# Autodesk Inventor assembly: wheel
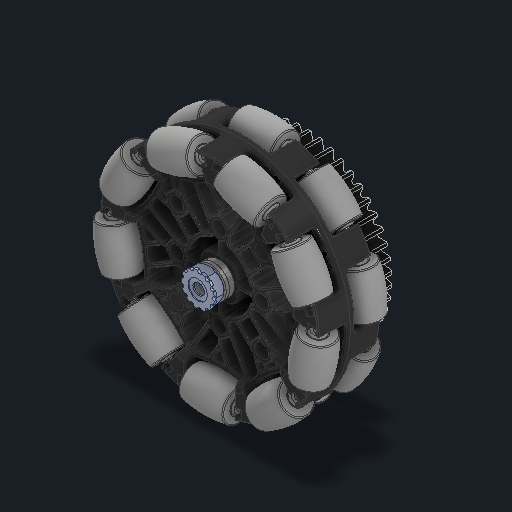
[picture p0: Inventor's stored thumbnail of the model, 512x512]
Saved by Autodesk Inventor 2024 (Build 280153000, 153)
## iProperties
Created: 2024-02-11
Part Number: wheel
Document SubType Name: Assembly
Designer: Averey Ku
Author: Averey Ku
## Documents named in this file (11)
- D:\vex_robotics\hardware\cad\vroomba_v0.1\chassis\drivebay\wheel.iam
- D:\vex_robotics\hardware\cad\VEX-CAD-Inventor-1.41\Motion\Wheels\Omni Wheel\2.75 Omni AS, No Insert.iam
- D:\vex_robotics\hardware\cad\VEX-CAD-Inventor-1.41\Motion\Wheels\Omni Wheel.iam
- D:\vex_robotics\hardware\cad\VEX-CAD-Inventor-1.41\Motion\Spacers\Spacer Nylon .375 OD\NSpacer .375 OD x .250.ipt
- D:\vex_robotics\hardware\cad\VEX-CAD-Inventor-1.41\Motion\Spacers\Spacer Nylon .375 OD.ipt
- D:\vex_robotics\hardware\cad\vroomba_v0.1\custom_parts\LS 48T Gear, No Insert.ipt
- D:\vex_robotics\hardware\cad\VEX-CAD-Inventor-1.41\Motion\Spacers\Washer Teflon\TWasher .375 OD x .04000.ipt
- D:\vex_robotics\hardware\cad\VEX-CAD-Inventor-1.41\Motion\Spacers\Washer Teflon.ipt
- D:\vex_robotics\hardware\cad\VEX-CAD-Inventor-1.41\Motion\Spacers\Washer Steel\SWasher .375 OD x .062500.ipt
- D:\vex_robotics\hardware\cad\VEX-CAD-Inventor-1.41\Motion\Spacers\Washer Steel.ipt
- D:\vex_robotics\hardware\cad\VEX-CAD-Inventor-1.41\Structure\Hardware\Nut Keps.ipt
## Components (7 placed, 6 different names)
1. 2.75 Omni AS, No Insert:1 [sub-assembly] — Insert:1, Insert:2, Insert:6
2. NSpacer .375 OD x .250:1 — Insert:1, Mate:1
3. NSpacer .375 OD x .250:2 — Insert:2, Insert:3
4. LS 48T Gear, No Insert:1 — Insert:3, Mate:1
5. TWasher .375 OD x .04000:1 — Insert:4, Insert:5
6. SWasher .375 OD x .062500:1 — Insert:4, Insert:6
7. Nut Keps:1 — Insert:5
## Relationships (7: Insert 6, Mate 1)
- Insert:1: 2.75 Omni AS, No Insert:1 ↔ NSpacer .375 OD x .250:1
- Insert:2: 2.75 Omni AS, No Insert:1 ↔ NSpacer .375 OD x .250:2
- Insert:3: NSpacer .375 OD x .250:2 ↔ LS 48T Gear, No Insert:1
- Mate:1: NSpacer .375 OD x .250:1 ↔ LS 48T Gear, No Insert:1
- Insert:4: TWasher .375 OD x .04000:1 ↔ SWasher .375 OD x .062500:1
- Insert:5: TWasher .375 OD x .04000:1 ↔ Nut Keps:1
- Insert:6: 2.75 Omni AS, No Insert:1 ↔ SWasher .375 OD x .062500:1
